# Autodesk Inventor assembly: Failed Assembly 1
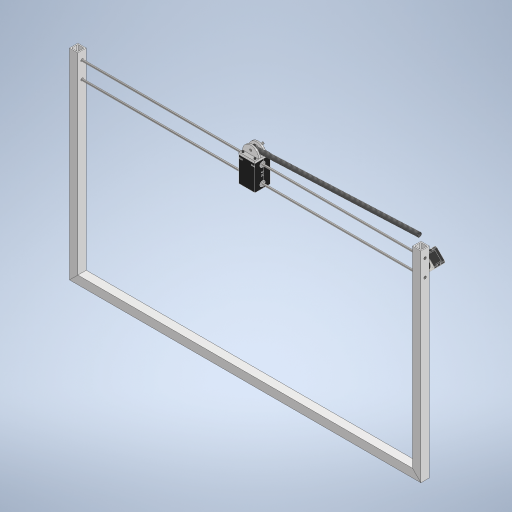
[picture p0: Inventor's stored thumbnail of the model, 512x512]
Saved by Autodesk Inventor 2023 (Build 270158000, 158)
## iProperties
Created: 2023-02-13
Part Number: Failed Assembly 1
Document SubType Name: Assembly
Designer: mbear
Author: mbear
## Documents named in this file (10)
- C:\Users\mbear\OneDrive\Documents\Inventor\Inverted Pendulum\Failed Assembly 1.iam
- C:\Users\mbear\OneDrive\Documents\Inventor\Inverted Pendulum\FrameAssembly.iam
- C:\Users\mbear\OneDrive\Documents\Inventor\Inverted Pendulum\NEMA17 Model.ipt
- C:\Users\mbear\OneDrive\Documents\Inventor\Inverted Pendulum\Carriage Assembly.iam
- C:\Users\mbear\OneDrive\Documents\Inventor\Inverted Pendulum\Pendulum Tubing.ipt
- C:\Users\mbear\OneDrive\Documents\Inventor\Inverted Pendulum\Linear Rod.ipt
- C:\Users\mbear\OneDrive\Documents\Inventor\Inverted Pendulum\Carriage Axle V1.ipt
- C:\Users\mbear\OneDrive\Documents\Inventor\Inverted Pendulum\M3 Square Nut.ipt
- C:\Users\mbear\OneDrive\Documents\Inventor\Inverted Pendulum\Hex_Socket_M3x16.ipt
- C:\Users\mbear\OneDrive\Documents\Inventor\Inverted Pendulum\M3 Nyloc Nut.ipt
## Components (17 placed, 9 different names)
1. FrameAssembly:1 [sub-assembly] — Insert:1, Insert:2, Insert:3, Insert:4
2. NEMA17 Model:1 — Insert:1, Insert:2
3. Carriage Assembly:2 [sub-assembly] — Mate:1, Mate:2, Insert:5, Insert:6, Angle:2, Insert:7, Angle:3, Insert:8, Angle:4, Insert:9, Angle:5, Insert:10, Insert:11, Insert:12, Insert:13
4. Linear Rod:1 — Insert:3, Mate:1
5. Linear Rod:2 — Insert:4, Mate:2
6. Carriage Axle V1:1 — Insert:5, Mate:3, Mate:4
7. Pendulum Tubing:1 — Mate:3, Mate:4, Mate:5, Flush:1
8. M3 Square Nut:1 — Insert:7, Angle:3
9. M3 Square Nut:2 — Insert:6, Angle:2
10. M3 Square Nut:3 — Insert:8, Angle:4
11. M3 Square Nut:4 — Insert:9, Angle:5
12. Hex_Socket_M3x16:1 — Insert:11
13. Hex_Socket_M3x16:2 — Insert:12
14. Hex_Socket_M3x16:3 — Insert:13
15. Hex_Socket_M3x16:4 — Insert:10
16. Hex_Socket_M3x16:5 — Mate:5, Insert:14, Flush:2
17. M3 Nyloc Nut:1 — Insert:14
## Relationships (25: Insert 14, Mate 5, Angle 4, Flush 2)
- Insert:1: FrameAssembly:1 ↔ NEMA17 Model:1
- Insert:2: FrameAssembly:1 ↔ NEMA17 Model:1
- Insert:3: FrameAssembly:1 ↔ Linear Rod:1
- Insert:4: FrameAssembly:1 ↔ Linear Rod:2
- Mate:1: Carriage Assembly:2 ↔ Linear Rod:1
- Mate:2: Carriage Assembly:2 ↔ Linear Rod:2
- Insert:5: Carriage Assembly:2 ↔ Carriage Axle V1:1
- Mate:3: Carriage Axle V1:1 ↔ Pendulum Tubing:1
- Mate:4: Carriage Axle V1:1 ↔ Pendulum Tubing:1
- Insert:6: Carriage Assembly:2 ↔ M3 Square Nut:2
- Angle:2 (0 deg): Carriage Assembly:2 ↔ M3 Square Nut:2
- Insert:7: Carriage Assembly:2 ↔ M3 Square Nut:1
- Angle:3 (0 deg): Carriage Assembly:2 ↔ M3 Square Nut:1
- Insert:8: Carriage Assembly:2 ↔ M3 Square Nut:3
- Angle:4 (0 deg): Carriage Assembly:2 ↔ M3 Square Nut:3
- Insert:9: Carriage Assembly:2 ↔ M3 Square Nut:4
- Angle:5 (0 deg): Carriage Assembly:2 ↔ M3 Square Nut:4
- Insert:10: Carriage Assembly:2 ↔ Hex_Socket_M3x16:4
- Insert:11: Carriage Assembly:2 ↔ Hex_Socket_M3x16:1
- Insert:12: Carriage Assembly:2 ↔ Hex_Socket_M3x16:2
- Insert:13: Carriage Assembly:2 ↔ Hex_Socket_M3x16:3
- Mate:5: Pendulum Tubing:1 ↔ Hex_Socket_M3x16:5
- Insert:14 (0.762 mm): Hex_Socket_M3x16:5 ↔ M3 Nyloc Nut:1
- Flush:1 (-6.35 mm): Pendulum Tubing:1
- Flush:2: Hex_Socket_M3x16:5
